# Autodesk Inventor assembly: 331-01
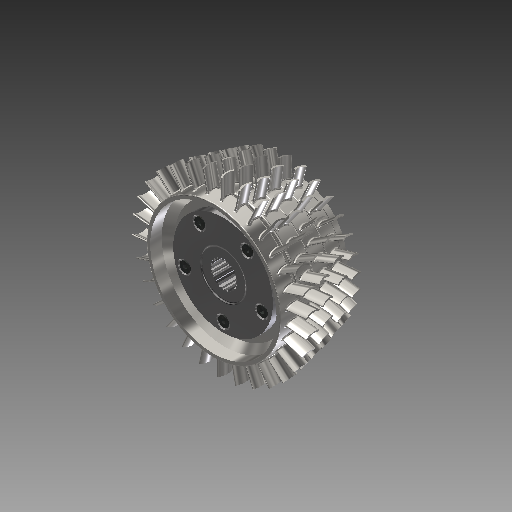
[picture p0: Inventor's stored thumbnail of the model, 512x512]
Saved by Autodesk Inventor 2019 (Build 230136000, 136)
## iProperties
Created: 2017-06-23
Part Number: 331-01
Document SubType Name: Assembly
Designer: t_crawk
Mass: 4347.38 g
Surface Area: 3209.51 cm^2
Volume: 888.272 cm^3
Density: 4.8942 g/cm^3
Author: t_crawk
## Documents named in this file (10)
- C:\TEMP\Jet Engine Model\Workspace\Rear Compression Assembly.iam
- C:\TEMP\Jet Engine Model\Workspace\Mid Axis Cover.ipt
- C:\TEMP\Jet Engine Model\Workspace\Rear Compression Link.ipt
- C:\TEMP\Jet Engine Model\Workspace\Mid Compression Fan.ipt
- C:\TEMP\Jet Engine Model\Workspace\Rear Compression Hub.ipt
- C:\TEMP\Jet Engine Model\Libraries\Content Center Files\en-US\ISO 10642(1)\ISO 10642 - M6 x  25.ipt
- C:\TEMP\Jet Engine Model\Workspace\Rear Compression Fan\Rear Compression Fan 01.ipt
- C:\Users\t_crawk\Documents\Inventor\Sample Files\Jet Engine\Main Axis\Rear Compression Fan.ipt
- C:\TEMP\Jet Engine Model\Workspace\Rear Compression Fan\Rear Compression Fan 02.ipt
- C:\TEMP\Jet Engine Model\Workspace\Rear Compression Fan\Rear Compression Fan 03.ipt
## Components (21 placed, 8 different names)
1. Mid Axis Cover:1 — Mate:1, Flush:1, Mate:2, Insert:1, Mate:4, Mate:5, Insert:6
2. Rear Compression Fan-01:1 — Mate:3, Mate:4, Mate:5, Mate:6, Insert:2
3. Rear Compression Fan-02:1 — Mate:6, Insert:2, Mate:7, Insert:3
4. Rear Compression Fan-03:1 — Mate:7, Insert:3, Mate:8, Insert:4
5. Mid Compression Fan:1 — Mate:8, Insert:4, Mate:9, Mate:11
6. Rear Compression Hub:1 — Mate:9, Mate:10, Insert:7, Mate:11
7. Rear Compression Link:1 — Insert:1, Mate:3, Mate:10
8. Rear Compression Link:2
9. Rear Compression Link:3
10. Rear Compression Link:4
11. Rear Compression Link:5
12. ISO 10642 M6 x  25:1 — Insert:6
13. ISO 10642 M6 x  25:2
14. ISO 10642 M6 x  25:3
15. ISO 10642 M6 x  25:4
16. ISO 10642 M6 x  25:5
17. ISO 10642 M6 x  25:6 — Insert:7
18. ISO 10642 M6 x  25:7
19. ISO 10642 M6 x  25:8
20. ISO 10642 M6 x  25:9
21. ISO 10642 M6 x  25:10
## Component patterns: (5 elements, first: Rear Compression Link:1), (5 elements, first: ISO 10642 M6 x  25:1), (5 elements, first: ISO 10642 M6 x  25:6)
## Relationships (18: Mate 11, Insert 6, Flush 1)
- Mate:1: Mid Axis Cover:1
- Flush:1: Mid Axis Cover:1
- Mate:2: Mid Axis Cover:1
- Insert:1: Mid Axis Cover:1 ↔ Rear Compression Link:1
- Mate:3: Rear Compression Fan-01:1 ↔ Rear Compression Link:1
- Mate:4: Mid Axis Cover:1 ↔ Rear Compression Fan-01:1
- Mate:5: Mid Axis Cover:1 ↔ Rear Compression Fan-01:1
- Mate:6: Rear Compression Fan-01:1 ↔ Rear Compression Fan-02:1
- Insert:2: Rear Compression Fan-01:1 ↔ Rear Compression Fan-02:1
- Mate:7: Rear Compression Fan-02:1 ↔ Rear Compression Fan-03:1
- Insert:3: Rear Compression Fan-02:1 ↔ Rear Compression Fan-03:1
- Mate:8: Rear Compression Fan-03:1 ↔ Mid Compression Fan:1
- Insert:4: Rear Compression Fan-03:1 ↔ Mid Compression Fan:1
- Mate:9: Mid Compression Fan:1 ↔ Rear Compression Hub:1
- Mate:10: Rear Compression Hub:1 ↔ Rear Compression Link:1
- Insert:6: Mid Axis Cover:1 ↔ ISO 10642 M6 x  25:1
- Insert:7: Rear Compression Hub:1 ↔ ISO 10642 M6 x  25:6
- Mate:11: Mid Compression Fan:1 ↔ Rear Compression Hub:1
